# Autodesk Inventor assembly: Box
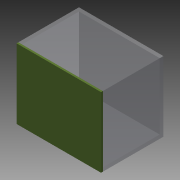
[picture p0: Inventor's stored thumbnail of the model, 180x180]
Saved by Autodesk Inventor 2013 (Build 170138000, 138)
## iProperties
Created: 2013-06-27
Part Number: Box
Document SubType Name: Assembly
Designer: Kyle
Author: Kyle
## Documents named in this file (3)
- C:\Users\Kyle\Documents\Inventor\2013\ROV\Box.iam
- C:\Users\Kyle\Documents\Inventor\2013\ROV\Box Bottom.ipt
- C:\Users\Kyle\Documents\Inventor\2013\ROV\Box Cover.ipt
## Components (2 placed, 2 different names)
1. Box Bottom:1 — Mate:1, Flush:1, Flush:2
2. Box Cover:1 — Mate:1, Flush:1, Flush:2
## Relationships (3: Flush 2, Mate 1)
- Mate:1: Box Bottom:1 ↔ Box Cover:1
- Flush:1: Box Bottom:1 ↔ Box Cover:1
- Flush:2: Box Bottom:1 ↔ Box Cover:1
